# Autodesk Inventor assembly: Whole Bot
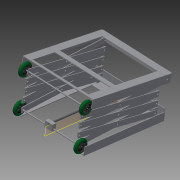
[picture p0: Inventor's stored thumbnail of the model, 180x180]
Saved by Autodesk Inventor 2015 (Build 190159000, 159)
## iProperties
Created: 2017-01-05
Part Number: Whole Bot
Document SubType Name: Assembly
Designer: ps2du
Author: ps2du
## Documents named in this file (8)
- E:\Robo Parts Inventor\Whole Bot.iam
- E:\Robo Parts Inventor\Bottom Assembly.iam
- E:\Robo Parts Inventor\Top Assembly.iam
- E:\Robo Parts Inventor\Scissor Lift.iam
- E:\Robo Parts Inventor\mockRod.ipt
- E:\Robo Parts Inventor\Vex Wheel.ipt
- E:\Robo Parts Inventor\coupler.ipt
- E:\Robo Parts Inventor\allthread.ipt
## Components (12 placed, 7 different names)
1. Bottom Assembly:1 [sub-assembly] — Rotational:1, Rotational:2, Cylindrical:15
2. Top Assembly:1 [sub-assembly] — Rotational:3
3. Scissor Lift:1 [sub-assembly] — Rotational:2, Rotational:6, Rotational:8
4. Scissor Lift:2 [sub-assembly] — Rotational:1, Rotational:3, Rotational:5, Rotational:7
5. mockRod:1 — Rotational:5, Rotational:6, Rotational:9, Rotational:10, Cylindrical:14
6. mockRod:2 — Rotational:7, Rotational:8, Rotational:11, Rotational:12
7. Vex Wheel:1 — Rotational:9
8. Vex Wheel:2 — Rotational:10
9. Vex Wheel:3 — Rotational:11
10. Vex Wheel:4 — Rotational:12
11. coupler:1 — Cylindrical:14, Rotational:13
12. allthread:1 — Rotational:13, Cylindrical:15
## Relationships (14: RevoluteJoint 12, CylindricalJoint 2)
- Rotational:1 [RevoluteJoint]: Bottom Assembly:1 ↔ Scissor Lift:2
- Rotational:2 [RevoluteJoint]: Bottom Assembly:1 ↔ Scissor Lift:1
- Rotational:3 [RevoluteJoint] (-34.925 mm): Top Assembly:1 ↔ Scissor Lift:2
- Rotational:5 [RevoluteJoint] (-22.225 mm): Scissor Lift:2 ↔ mockRod:1
- Rotational:6 [RevoluteJoint] (-22.225 mm): Scissor Lift:1 ↔ mockRod:1
- Rotational:7 [RevoluteJoint] (-25.4 mm): Scissor Lift:2 ↔ mockRod:2
- Rotational:8 [RevoluteJoint] (-25.4 mm): Scissor Lift:1 ↔ mockRod:2
- Rotational:9 [RevoluteJoint]: mockRod:1 ↔ Vex Wheel:1
- Rotational:10 [RevoluteJoint]: mockRod:1 ↔ Vex Wheel:2
- Rotational:11 [RevoluteJoint]: mockRod:2 ↔ Vex Wheel:3
- Rotational:12 [RevoluteJoint]: mockRod:2 ↔ Vex Wheel:4
- Cylindrical:14: mockRod:1 ↔ coupler:1
- Rotational:13 [RevoluteJoint]: coupler:1 ↔ allthread:1
- Cylindrical:15: Bottom Assembly:1 ↔ allthread:1
